# Autodesk Inventor assembly: Assieme_Struttura
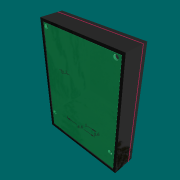
[picture p0: Inventor's stored thumbnail of the model, 180x180]
Saved by Autodesk Inventor 2020 (Build 240168000, 168)
## iProperties
Created: 2025-02-23
Part Number: Assieme_Struttura
Document SubType Name: Assembly
Designer: Nicola Milia
Author: Nicola Milia
## Documents named in this file (4)
- C:\Users\milit\Desktop\Progetti\Project THOR\Coperchio Dx V3\Assieme_Struttura.iam
- C:\Users\milit\Desktop\Progetti\Project THOR\Coperchio Dx V3\PCB.ipt
- C:\Users\milit\Desktop\Progetti\Project THOR\Coperchio Dx V3\struttura.ipt
- C:\Users\milit\Desktop\Progetti\Project THOR\Coperchio Dx V3\tappo_superiore.ipt
## Components (3 placed, 3 different names)
1. PCB:1 — Allineato:1, Allineato:2
2. struttura:1 — Allineato:1, Allineato:2, Allineato:3, Allineato:4, Allineato:5, Allineato:6
3. tappo_superiore:1 — Allineato:3, Allineato:4, Allineato:5, Allineato:6
## Relationships (6: Flush 6)
- Allineato:1 [Flush]: PCB:1 ↔ struttura:1
- Allineato:2 [Flush]: PCB:1 ↔ struttura:1
- Allineato:3 [Flush]: struttura:1 ↔ tappo_superiore:1
- Allineato:4 [Flush]: struttura:1 ↔ tappo_superiore:1
- Allineato:5 [Flush]: struttura:1 ↔ tappo_superiore:1
- Allineato:6 [Flush]: struttura:1 ↔ tappo_superiore:1
